# Autodesk Inventor assembly: XPulleySupport
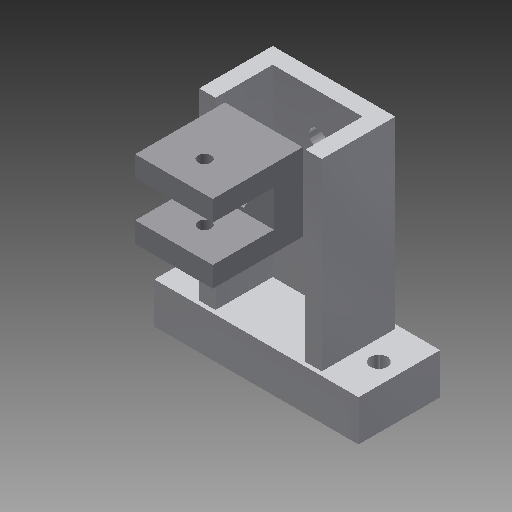
[picture p0: Inventor's stored thumbnail of the model, 512x512]
Saved by Autodesk Inventor 2019 (Build 230136000, 136)
## iProperties
Created: 2019-08-19
Part Number: XPulleySupport
Document SubType Name: Assembly
Designer: Bruno
Author: Bruno
## Documents named in this file (3)
- C:\Users\Bruno\Stuff\TPINFO\tp-info\XPulleySupport.iam
- C:\Users\Bruno\Stuff\TPINFO\tp-info\XPulleySupportBase.ipt
- C:\Users\Bruno\Stuff\TPINFO\tp-info\XPulleySupportHolder.ipt
## Components (2 placed, 2 different names)
1. XPulleySupportBase:1 — Cylindrical:1, Angle:1
2. XPulleySupportHolder:1 — Cylindrical:1, Angle:1
## Relationships (2: CylindricalJoint 1, Angle 1)
- Cylindrical:1: XPulleySupportBase:1 ↔ XPulleySupportHolder:1
- Angle:1 (0 deg): XPulleySupportBase:1 ↔ XPulleySupportHolder:1
